# Autodesk Inventor assembly: actuator assembly
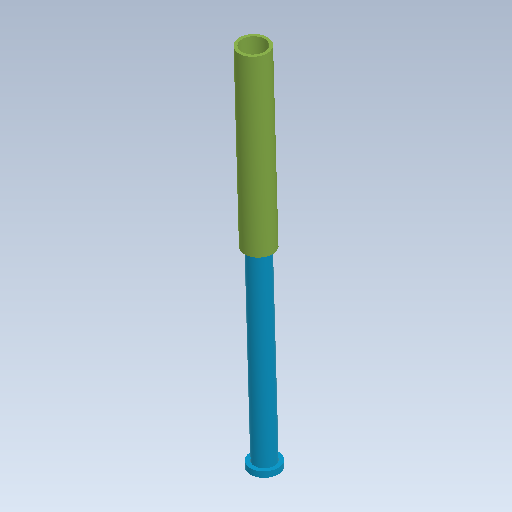
[picture p0: Inventor's stored thumbnail of the model, 512x512]
Saved by Autodesk Inventor 2020 (Build 240168000, 168)
## iProperties
Created: 2020-12-11
Part Number: actuator assembly
Document SubType Name: Assembly
Designer: Vikki
Author: Vikki
## Documents named in this file (3)
- D:\borewell rescuebot\pll manipulator files\sps manipulator\actuator assembly.iam
- D:\borewell rescuebot\pll manipulator files\sps manipulator\piston.ipt
- D:\borewell rescuebot\pll manipulator files\sps manipulator\plunger.ipt
## Components (2 placed, 2 different names)
1. piston:1
2. plunger:1
## Relationships (1: Mate 1)
- [Mate]: piston:1 ↔ plunger:1
